# Autodesk Inventor assembly: Lidarv4
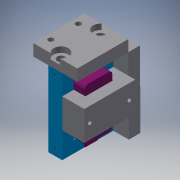
[picture p0: Inventor's stored thumbnail of the model, 180x180]
Saved by Autodesk Inventor 2019 (Build 230136000, 136)
## iProperties
Created: 2020-08-15
Part Number: Lidarv4
Document SubType Name: Assembly
Designer: james
Author: james
## Documents named in this file (6)
- F:\JimsRobot\FIRSTRobots\Design\Library\Jims\Lidarv4.iam
- F:\JimsRobot\FIRSTRobots\Design\Library\Jims\LidarV4Mount.ipt
- F:\JimsRobot\FIRSTRobots\Design\Library\Garmin\LIDAR-LITE V4.ipt
- F:\JimsRobot\FIRSTRobots\Design\Library\Jims\LidarV4MountBack.ipt
- F:\JimsRobot\FIRSTRobots\Design\Library\Jims\LidarV4MountLongPlate.ipt
- F:\JimsRobot\FIRSTRobots\Design\Library\Jims\LidarV4MountShortPlate.ipt
## Components (5 placed, 5 different names)
1. LidarV4Mount:1 — Mate:1, Mate:2, Flush:1, Mate:3, Mate:4, Mate:5, Mate:6, Mate:7, Mate:8
2. LIDAR-LITE V4:1 — Mate:1, Mate:2, Flush:1
3. LidarV4MountBack:1 — Mate:3, Mate:4
4. LidarV4MountLongPlate:1 — Mate:5, Mate:6
5. LidarV4MountShortPlate:1 — Mate:7, Mate:8
## Relationships (9: Mate 8, Flush 1)
- Mate:1: LidarV4Mount:1 ↔ LIDAR-LITE V4:1
- Mate:2: LidarV4Mount:1 ↔ LIDAR-LITE V4:1
- Flush:1: LidarV4Mount:1 ↔ LIDAR-LITE V4:1
- Mate:3: LidarV4Mount:1 ↔ LidarV4MountBack:1
- Mate:4: LidarV4Mount:1 ↔ LidarV4MountBack:1
- Mate:5: LidarV4Mount:1 ↔ LidarV4MountLongPlate:1
- Mate:6: LidarV4Mount:1 ↔ LidarV4MountLongPlate:1
- Mate:7: LidarV4Mount:1 ↔ LidarV4MountShortPlate:1
- Mate:8: LidarV4Mount:1 ↔ LidarV4MountShortPlate:1
